# Autodesk Inventor assembly: FreundBumper
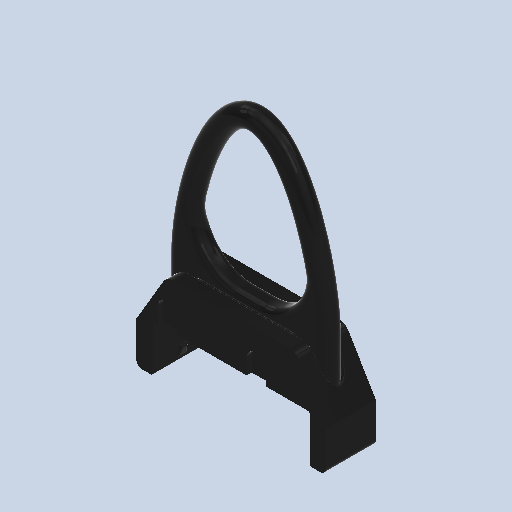
[picture p0: Inventor's stored thumbnail of the model, 512x512]
Saved by Autodesk Inventor 2022.4 (Build 264492000, 492)
## iProperties
Created: 2021-10-10
Part Number: FreundBumper
Document SubType Name: Assembly
Designer: t-nagamine
Mass: 18.4899 g
Surface Area: 86.5115 cm^2
Volume: 14.4452 cm^3
Density: 1.28 g/cm^3
Author: t-nagamine
## Documents named in this file (3)
- C:\Users\supra\Documents\GitHub\OpenPlatform_ver3_0\UpperBody\Trunk\FreundBumper.iam
- C:\Users\supra\Documents\GitHub\OpenPlatform_ver3_0\UpperBody\Trunk\FreundBumper_Stand.ipt
- C:\Users\supra\Documents\GitHub\OpenPlatform_ver3_0\UpperBody\Trunk\FrontBumper_main.ipt
## Components (2 placed, 2 different names)
1. FreundBumper_Stand:1 — 挿入:1, メイト:1
2. FrontBumper_main:1 — 挿入:1, メイト:1
## Relationships (2: Insert 1, Mate 1)
- 挿入:1 [Insert]: FreundBumper_Stand:1 ↔ FrontBumper_main:1
- メイト:1 [Mate]: FreundBumper_Stand:1 ↔ FrontBumper_main:1
